# Autodesk Inventor assembly: UpperBackLink
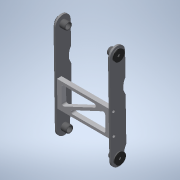
[picture p0: Inventor's stored thumbnail of the model, 180x180]
Saved by Autodesk Inventor 2020.4 (Build 244396000, 396)
## iProperties
Created: 2016-08-23
Part Number: UpperBackLink
Material: 一般
Document SubType Name: Assembly
Designer: hiro
Mass: 25.265 g
Surface Area: 146.992 cm^2
Volume: 11.3922 cm^3
Density: 2.21774 g/cm^3
Author: hiro
## Documents named in this file (5)
- C:\Users\Masato\Documents\Inventor\CIT Brains_Inventor\OpenPlatform_ver3_0\下半身\リンク\UpperBackLink.iam
- C:\Users\Masato\Documents\Inventor\CIT Brains_Inventor\OpenPlatform_ver3_0\下半身\リンク\リンク_メインフレーム_6_1.ipt
- C:\Users\Masato\Documents\Inventor\CIT Brains_Inventor\OpenPlatform_ver3_0\下半身\リンク\リンク_ふくらはぎ_サブフレーム_1_2.ipt
- C:\Users\Masato\Documents\Inventor\CIT Brains_Inventor\OpenPlatform_ver3_0\Ready_Made\80F-0608.ipt
- C:\Users\Masato\Documents\Inventor\CIT Brains_Inventor\OpenPlatform_ver3_0\Ready_Made\UUW-0312-10BH.ipt
## Components (11 placed, 4 different names)
1. リンク_メインフレーム_6_1:1 — 挿入:14, 挿入:16, 挿入:21, 挿入:22
2. リンク_メインフレーム_6_1:2 — 挿入:13, 挿入:15, 挿入:23, 挿入:24
3. 80F-0608:1 — 挿入:13, 挿入:20
4. 80F-0608:2 — 挿入:14, 挿入:18
5. 80F-0608:3 — 挿入:15, 挿入:19
6. 80F-0608:4 — 挿入:16, 挿入:17
7. UUW-0312-10BH:1 — 挿入:17
8. UUW-0312-10BH:2 — 挿入:18
9. UUW-0312-10BH:3 — 挿入:20
10. UUW-0312-10BH:4 — 挿入:19
11. リンク_ふくらはぎ_サブフレーム_1_2:1 — 挿入:21, 挿入:22, 挿入:23, 挿入:24
## Relationships (12: Insert 12)
- 挿入:13 [Insert]: リンク_メインフレーム_6_1:2 ↔ 80F-0608:1
- 挿入:14 [Insert]: リンク_メインフレーム_6_1:1 ↔ 80F-0608:2
- 挿入:15 [Insert]: リンク_メインフレーム_6_1:2 ↔ 80F-0608:3
- 挿入:16 [Insert]: リンク_メインフレーム_6_1:1 ↔ 80F-0608:4
- 挿入:17 [Insert]: 80F-0608:4 ↔ UUW-0312-10BH:1
- 挿入:18 [Insert]: 80F-0608:2 ↔ UUW-0312-10BH:2
- 挿入:19 [Insert]: 80F-0608:3 ↔ UUW-0312-10BH:4
- 挿入:20 [Insert]: 80F-0608:1 ↔ UUW-0312-10BH:3
- 挿入:21 [Insert]: リンク_メインフレーム_6_1:1 ↔ リンク_ふくらはぎ_サブフレーム_1_2:1
- 挿入:22 [Insert]: リンク_メインフレーム_6_1:1 ↔ リンク_ふくらはぎ_サブフレーム_1_2:1
- 挿入:23 [Insert]: リンク_メインフレーム_6_1:2 ↔ リンク_ふくらはぎ_サブフレーム_1_2:1
- 挿入:24 [Insert]: リンク_メインフレーム_6_1:2 ↔ リンク_ふくらはぎ_サブフレーム_1_2:1
